# Autodesk Inventor assembly: Ensamblaje
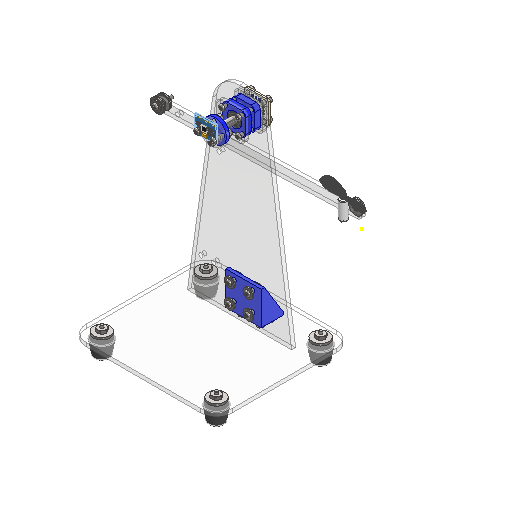
[picture p0: Inventor's stored thumbnail of the model, 512x512]
Saved by Autodesk Inventor 2025.3 (Build 293356000, 356)
## iProperties
Created: 2025-11-11
Part Number: Ensamblaje
Document SubType Name: Assembly
Designer: Gabriel Bojaca
Author: Gabriel Bojaca
## Documents named in this file (28)
- C:\Users\Gabriel Bojaca\Documents\Inventor\TDC\Ensamblaje.iam
- C:\Users\Gabriel Bojaca\Documents\Inventor\TDC\Acople_eje.ipt
- C:\Users\Gabriel Bojaca\Documents\Inventor\TDC\Base.ipt
- C:\Users\Gabriel Bojaca\Documents\Inventor\TDC\Chumacera.ipt
- C:\Users\Gabriel Bojaca\Documents\Inventor\TDC\Columna.ipt
- C:\Users\Gabriel Bojaca\Documents\Inventor\TDC\Escuadra.ipt
- C:\Users\Gabriel Bojaca\Documents\Inventor\TDC\Tope_rodamiento.ipt
- C:\Users\Gabriel Bojaca\Documents\Inventor\TDC\MR126ZZ-6x12x4mm.ipt
- C:\Users\Gabriel Bojaca\Documents\Inventor\TDC\Pendulo.ipt
- C:\Users\Gabriel Bojaca\Documents\Inventor\TDC\eje.ipt
- C:\Users\Gabriel Bojaca\Documents\Inventor\TDC\AS5600_magnetic_encoder\AS5600_magnetic_encoder\AS5600_magnetic_encoder.ipt
- C:\Users\Gabriel Bojaca\Documents\Inventor\TDC\Separador.ipt
- C:\Users\Gabriel Bojaca\Documents\Inventor\TDC\iman.ipt
- C:\Users\Gabriel Bojaca\Documents\Inventor\TDC\MPU_6050\MPU_6050\MPU_6050.ipt
- C:\Users\Gabriel Bojaca\Documents\Inventor\TDC\Coreless_Motor_716\Coreless_Motor_716\Coreless_Motor_716.ipt
- C:\Users\Gabriel Bojaca\Documents\Inventor\Content Center Files\R2025\en-US\ANSI B18.3.4M(1)\ANSI B18.3.4M - M3 x 0.5 x 30(2).ipt
- C:\Users\Gabriel Bojaca\Documents\Inventor\Content Center Files\R2025\en-US\ANSI B18.2.4.2M\ANSI B18.2.4.2M - M3x0,5 - 5,5.ipt
- C:\Users\Gabriel Bojaca\Documents\Inventor\Content Center Files\R2025\en-US\ANSI B18.3.4M(1)\ANSI B18.3.4M - M3 x 0.5 x 10(2).ipt
- C:\Users\Gabriel Bojaca\Documents\Inventor\Content Center Files\R2025\en-US\ANSI B18.3.4M(1)\ANSI B18.3.4M - M3 x 0.5 x 16(2).ipt
- C:\Users\Gabriel Bojaca\Documents\Inventor\TDC\Arandela_3_16.ipt
- C:\Users\Gabriel Bojaca\Documents\Inventor\TDC\Arandela_1_8.ipt
- C:\Users\Gabriel Bojaca\Documents\Inventor\TDC\Tuerca_M3.ipt
- C:\Users\Gabriel Bojaca\Documents\Inventor\Content Center Files\R2025\en-US\ANSI B18.3.4M(1)\ANSI B18.3.4M - M3 x 0.5 x 12(2).ipt
- C:\Users\Gabriel Bojaca\Documents\Inventor\TDC\Patas_para_licuadora.ipt
- C:\Users\Gabriel Bojaca\Documents\Inventor\Content Center Files\R2025\en-US\ANSI B18.6.3(48)\ANSI B18.6.3 - 4-40 x 3_4(7).ipt
- C:\Users\Gabriel Bojaca\Documents\Inventor\Content Center Files\R2025\en-US\ANSI B18.2.2(06)\ANSI B18.2.2 - 5 - 44(06).ipt
- C:\Users\Gabriel Bojaca\Documents\Inventor\Content Center Files\R2025\en-US\ASTM F436(1)\ASTM F436 - 1_4(1).ipt
- C:\Users\Gabriel Bojaca\Documents\Inventor\TDC\PROPELLER - 8x4.5 CW\cw_2blades.ipt
## Components (90 placed, 27 different names)
1. Acople_eje:1 — Mate:26, Mate:27, Mate:28, Mate:29, Mate:74, Mate:76, Mate:77, Mate:81, Mate:86
2. Base:1 — Mate:1, Mate:8, Mate:9, Mate:10, Mate:144, Mate:153, Mate:154, Mate:155, Mate:156, Mate:157, Mate:158, Mate:159, Mate:162, Mate:175, Mate:176, Mate:177, Mate:179, Mate:180, Mate:183
3. Chumacera:1 — Mate:12, Flush:1, Mate:16, Mate:20, Mate:22
4. Columna:1 — Mate:5, Mate:6, Mate:7, Mate:13, Mate:14, Mate:15, Mate:16, Mate:54, Mate:115, Mate:133, Mate:134, Mate:135, Mate:136
5. Escuadra:1 — Mate:5, Mate:6, Mate:7, Mate:8, Mate:9, Mate:10, Mate:116, Mate:117, Mate:137, Mate:142, Mate:143, Mate:148, Mate:149, Mate:150, Mate:151, Mate:152
6. Tope_rodamiento:1 — Mate:20, Mate:21, Mate:22, Mate:23, Mate:54, Mate:55, Mate:56, Mate:62, Mate:63, Mate:65, Mate:66, Mate:69, Mate:70
7. Chumacera:2 — Mate:11, Flush:2, Mate:15, Mate:18, Mate:19
8. MR126ZZ-6x12x4mm:1 — Mate:12, Flush:1, Mate:13, Mate:21, Mate:31
9. MR126ZZ-6x12x4mm:2 — Mate:11, Flush:2, Mate:14, Mate:17
10. Tope_rodamiento:2 — Mate:17, Mate:18, Mate:19, Mate:23, Mate:32, Mate:33, Mate:34, Mate:35, Mate:36, Mate:37, Mate:38, Mate:39, Mate:40, Mate:41
11. Pendulo:1 — Mate:26, Mate:27, Mate:28, Mate:30, Mate:46, Mate:47, Mate:48, Mate:49, Mate:186, Mate:53, Mate:72, Mate:73, Mate:78, Mate:87, Mate:94, Mate:95, Mate:96, Mate:108, Mate:109
12. eje:1 — Mate:29, Mate:30, Mate:31, Mate:43, Mate:44
13. AS5600_magnetic_encoder:1 — Mate:32, Mate:33, Mate:42, Mate:45, Mate:58, Mate:64, Mate:67, Mate:68
14. Separador:1 — Mate:35, Mate:40
15. Separador:2 — Mate:36, Mate:41, Mate:42
16. Separador:3 — Mate:34, Mate:38
17. Separador:4 — Mate:37, Mate:39
18. iman:1 — Mate:43, Mate:44, Mate:45
19. MPU_6050:1 — Mate:50, Mate:51, Mate:52, Mate:80, Mate:82, Mate:84, Mate:85
20. Separador:5 — Mate:46, Mate:48, Mate:50, Mate:52
21. Separador:6 — Mate:47, Mate:49, Mate:51
22. Coreless_Motor_716:1 — Mate:186, Mate:53, Mate:87, Mate:184, Mate:185
23. Broached Hexagon Socket Button Head Cap Screw - Metric M3 x 0.5 x 30:2 — Mate:55, Mate:56, Mate:57
24. ANSI B18.2.4.2M M3x0,5:1 — Mate:57, Mate:58
25. Broached Hexagon Socket Button Head Cap Screw - Metric M3 x 0.5 x 30:3 — Mate:69, Mate:70
26. ANSI B18.2.4.2M M3x0,5:2 — Mate:68
27. Broached Hexagon Socket Button Head Cap Screw - Metric M3 x 0.5 x 30:4 — Mate:62, Mate:63
28. ANSI B18.2.4.2M M3x0,5:3 — Mate:64
29. Broached Hexagon Socket Button Head Cap Screw - Metric M3 x 0.5 x 30:5 — Mate:65, Mate:66
30. ANSI B18.2.4.2M M3x0,5:4 — Mate:67
31. Broached Hexagon Socket Button Head Cap Screw - Metric M3 x 0.5 x 10:1 — Mate:72, Mate:73
32. ANSI B18.2.4.2M M3x0,5:5 — Mate:74
33. Broached Hexagon Socket Button Head Cap Screw - Metric M3 x 0.5 x 10:2 — Mate:76, Mate:78
34. ANSI B18.2.4.2M M3x0,5:6 — Mate:77
35. Broached Hexagon Socket Button Head Cap Screw - Metric M3 x 0.5 x 16:1 — Mate:80, Mate:82
36. ANSI B18.2.4.2M M3x0,5:7 — Mate:81
37. Broached Hexagon Socket Button Head Cap Screw - Metric M3 x 0.5 x 16:2 — Mate:84, Mate:85
38. ANSI B18.2.4.2M M3x0,5:8 — Mate:86
39. Broached Hexagon Socket Button Head Cap Screw - Metric M3 x 0.5 x 16:3 — Mate:88, Mate:89, Mate:91, Mate:93, Mate:94, Mate:97, Mate:98, Mate:101, Mate:102
40. Arandela_3_16:1 — Mate:96, Mate:97, Mate:99
41. Arandela_1_8:1 — Mate:100, Mate:101, Mate:103
42. Arandela_3_16:2 — Mate:89, Mate:90, Mate:92
43. Arandela_1_8:2 — Mate:88, Mate:90, Mate:91
44. Tuerca_M3:2 — Mate:102, Mate:103
45. Arandela_3_16:3 — Mate:98, Mate:99, Mate:100
46. Arandela_3_16:4 — Mate:92, Mate:93, Mate:95
47. Arandela_3_16:5 — Mate:104, Mate:106, Mate:108, Mate:109
48. Arandela_3_16:6 — Mate:104, Mate:105, Mate:107
49. Arandela_3_16:7 — Mate:105, Mate:106, Mate:107
50. Broached Hexagon Socket Button Head Cap Screw - Metric M3 x 0.5 x 12:1 — Mate:117
51. Arandela_1_8:3 — Mate:116
52. Arandela_1_8:4 — Mate:115
53. Tuerca_M3:3
54. Broached Hexagon Socket Button Head Cap Screw - Metric M3 x 0.5 x 12:2 — Mate:134
55. Arandela_1_8:5 — Flush:6, Mate:137
56. Arandela_1_8:6 — Flush:4, Mate:133
57. Tuerca_M3:4
58. Broached Hexagon Socket Button Head Cap Screw - Metric M3 x 0.5 x 12:3 — Mate:135
59. Arandela_1_8:7 — Flush:6, Flush:7
60. Arandela_1_8:8 — Flush:4, Flush:5
61. Tuerca_M3:5
62. Broached Hexagon Socket Button Head Cap Screw - Metric M3 x 0.5 x 12:4 — Mate:136
63. Arandela_1_8:9 — Flush:7
64. Arandela_1_8:10 — Flush:5
65. Tuerca_M3:6
66. Broached Hexagon Socket Button Head Cap Screw - Metric M3 x 0.5 x 10:3 — Mate:142, Mate:143
67. Tuerca_M3:7 — Mate:144
68. Broached Hexagon Socket Button Head Cap Screw - Metric M3 x 0.5 x 10:4 — Mate:148, Mate:149
69. Tuerca_M3:8 — Flush:9, Flush:10
70. Broached Hexagon Socket Button Head Cap Screw - Metric M3 x 0.5 x 10:5 — Flush:8, Mate:150, Mate:152
71. Tuerca_M3:9 — Flush:9
72. Broached Hexagon Socket Button Head Cap Screw - Metric M3 x 0.5 x 10:6 — Flush:8, Mate:151
73. Tuerca_M3:10 — Flush:10, Mate:153
74. Patas_para_licuadora:1 — Mate:154, Mate:155
75. Patas_para_licuadora:2 — Mate:156, Flush:11, Mate:160, Mate:161
76. Patas_para_licuadora:3 — Mate:157, Flush:12, Mate:159, Mate:182
77. Patas_para_licuadora:4 — Mate:158, Flush:11, Flush:12, Mate:181
78. Slotted Hex Head Machine Screw - Inch 4-40 x 3/4:1 — Mate:160, Mate:161, Mate:163, Mate:165
79. Hex Machine Screw Nut - Inch 5 - 44:1 — Mate:164, Mate:165
80. Circular Washer (Inch) 1/4:1 — Mate:162, Mate:163, Mate:164
81. Slotted Hex Head Machine Screw - Inch 4-40 x 3/4:2 — Mate:175, Mate:182
82. Hex Machine Screw Nut - Inch 5 - 44:2
83. Circular Washer (Inch) 1/4:2 — Mate:183
84. Slotted Hex Head Machine Screw - Inch 4-40 x 3/4:3 — Flush:14, Mate:177, Mate:181
85. Hex Machine Screw Nut - Inch 5 - 44:3
86. Circular Washer (Inch) 1/4:3 — Mate:179
87. Slotted Hex Head Machine Screw - Inch 4-40 x 3/4:4 — Flush:14, Mate:176
88. Hex Machine Screw Nut - Inch 5 - 44:4
89. Circular Washer (Inch) 1/4:4 — Mate:180
90. cw_2blades:1 — Mate:184, Mate:185
## Relationships (189: Mate 177, Flush 12)
- Mate:1: Base:1
- Mate:5: Columna:1 ↔ Escuadra:1
- Mate:6: Columna:1 ↔ Escuadra:1
- Mate:7: Columna:1 ↔ Escuadra:1
- Mate:8: Base:1 ↔ Escuadra:1
- Mate:9: Base:1 ↔ Escuadra:1
- Mate:10: Base:1 ↔ Escuadra:1
- Mate:11: Chumacera:2 ↔ MR126ZZ-6x12x4mm:2
- Mate:12: Chumacera:1 ↔ MR126ZZ-6x12x4mm:1
- Flush:1 (0.5 mm): Chumacera:1 ↔ MR126ZZ-6x12x4mm:1
- Flush:2 (-0.5 mm): Chumacera:2 ↔ MR126ZZ-6x12x4mm:2
- Mate:13: Columna:1 ↔ MR126ZZ-6x12x4mm:1
- Mate:14: Columna:1 ↔ MR126ZZ-6x12x4mm:2
- Mate:15: Columna:1 ↔ Chumacera:2
- Mate:16: Chumacera:1 ↔ Columna:1
- Mate:17: MR126ZZ-6x12x4mm:2 ↔ Tope_rodamiento:2
- Mate:18: Chumacera:2 ↔ Tope_rodamiento:2
- Mate:19: Chumacera:2 ↔ Tope_rodamiento:2
- Mate:20: Chumacera:1 ↔ Tope_rodamiento:1
- Mate:21: Tope_rodamiento:1 ↔ MR126ZZ-6x12x4mm:1
- Mate:22: Chumacera:1 ↔ Tope_rodamiento:1
- Mate:23: Tope_rodamiento:1 ↔ Tope_rodamiento:2
- Mate:26: Acople_eje:1 ↔ Pendulo:1
- Mate:27: Acople_eje:1 ↔ Pendulo:1
- Mate:28: Acople_eje:1 ↔ Pendulo:1
- Mate:29: Acople_eje:1 ↔ eje:1
- Mate:30: Pendulo:1 ↔ eje:1
- Mate:31: MR126ZZ-6x12x4mm:1 ↔ eje:1
- Mate:32: Tope_rodamiento:2 ↔ AS5600_magnetic_encoder:1
- Mate:33: Tope_rodamiento:2 ↔ AS5600_magnetic_encoder:1
- Mate:34: Tope_rodamiento:2 ↔ Separador:3
- Mate:35: Tope_rodamiento:2 ↔ Separador:1
- Mate:36: Tope_rodamiento:2 ↔ Separador:2
- Mate:37: Tope_rodamiento:2 ↔ Separador:4
- Mate:38: Tope_rodamiento:2 ↔ Separador:3
- Mate:39: Tope_rodamiento:2 ↔ Separador:4
- Mate:40: Tope_rodamiento:2 ↔ Separador:1
- Mate:41: Tope_rodamiento:2 ↔ Separador:2
- Mate:42: AS5600_magnetic_encoder:1 ↔ Separador:2
- Mate:43: eje:1 ↔ iman:1
- Mate:44: eje:1 ↔ iman:1
- Mate:45 (0.5 mm): AS5600_magnetic_encoder:1 ↔ iman:1
- Mate:46: Pendulo:1 ↔ Separador:5
- Mate:47: Pendulo:1 ↔ Separador:6
- Mate:48: Pendulo:1 ↔ Separador:5
- Mate:49: Pendulo:1 ↔ Separador:6
- Mate:50: MPU_6050:1 ↔ Separador:5
- Mate:51: MPU_6050:1 ↔ Separador:6
- Mate:52: MPU_6050:1 ↔ Separador:5
- Mate:186 (-13 mm): Pendulo:1 ↔ Coreless_Motor_716:1
- Mate:53 (3.5 mm): Pendulo:1 ↔ Coreless_Motor_716:1
- Mate:54: Columna:1 ↔ Tope_rodamiento:1
- Mate:55: Tope_rodamiento:1 ↔ Broached Hexagon Socket Button Head Cap Screw - Metric M3 x 0.5 x 30:2
- Mate:56: Tope_rodamiento:1 ↔ Broached Hexagon Socket Button Head Cap Screw - Metric M3 x 0.5 x 30:2
- Mate:57: Broached Hexagon Socket Button Head Cap Screw - Metric M3 x 0.5 x 30:2 ↔ ANSI B18.2.4.2M M3x0,5:1
- Mate:58: AS5600_magnetic_encoder:1 ↔ ANSI B18.2.4.2M M3x0,5:1
- [Mate]: Broached Hexagon Socket Button Head Cap Screw - Metric M3 x 0.5 x 30:3 ↔ ANSI B18.2.4.2M M3x0,5:2
- [Mate]: Broached Hexagon Socket Button Head Cap Screw - Metric M3 x 0.5 x 30:4 ↔ ANSI B18.2.4.2M M3x0,5:3
- [Mate]: Broached Hexagon Socket Button Head Cap Screw - Metric M3 x 0.5 x 30:5 ↔ ANSI B18.2.4.2M M3x0,5:4
- Mate:62: Tope_rodamiento:1 ↔ Broached Hexagon Socket Button Head Cap Screw - Metric M3 x 0.5 x 30:4
- Mate:63: Tope_rodamiento:1 ↔ Broached Hexagon Socket Button Head Cap Screw - Metric M3 x 0.5 x 30:4
- Mate:64: AS5600_magnetic_encoder:1 ↔ ANSI B18.2.4.2M M3x0,5:3
- Mate:65: Tope_rodamiento:1 ↔ Broached Hexagon Socket Button Head Cap Screw - Metric M3 x 0.5 x 30:5
- Mate:66: Tope_rodamiento:1 ↔ Broached Hexagon Socket Button Head Cap Screw - Metric M3 x 0.5 x 30:5
- Mate:67: AS5600_magnetic_encoder:1 ↔ ANSI B18.2.4.2M M3x0,5:4
- Mate:68: AS5600_magnetic_encoder:1 ↔ ANSI B18.2.4.2M M3x0,5:2
- Mate:69: Tope_rodamiento:1 ↔ Broached Hexagon Socket Button Head Cap Screw - Metric M3 x 0.5 x 30:3
- Mate:70: Tope_rodamiento:1 ↔ Broached Hexagon Socket Button Head Cap Screw - Metric M3 x 0.5 x 30:3
- [Mate]: Broached Hexagon Socket Button Head Cap Screw - Metric M3 x 0.5 x 10:1 ↔ ANSI B18.2.4.2M M3x0,5:5
- Mate:72: Pendulo:1 ↔ Broached Hexagon Socket Button Head Cap Screw - Metric M3 x 0.5 x 10:1
- Mate:73: Pendulo:1 ↔ Broached Hexagon Socket Button Head Cap Screw - Metric M3 x 0.5 x 10:1
- Mate:74: Acople_eje:1 ↔ ANSI B18.2.4.2M M3x0,5:5
- [Mate]: Broached Hexagon Socket Button Head Cap Screw - Metric M3 x 0.5 x 10:2 ↔ ANSI B18.2.4.2M M3x0,5:6
- Mate:76: Acople_eje:1 ↔ Broached Hexagon Socket Button Head Cap Screw - Metric M3 x 0.5 x 10:2
- Mate:77: Acople_eje:1 ↔ ANSI B18.2.4.2M M3x0,5:6
- Mate:78: Pendulo:1 ↔ Broached Hexagon Socket Button Head Cap Screw - Metric M3 x 0.5 x 10:2
- [Mate]: Broached Hexagon Socket Button Head Cap Screw - Metric M3 x 0.5 x 16:1 ↔ ANSI B18.2.4.2M M3x0,5:7
- Mate:80: MPU_6050:1 ↔ Broached Hexagon Socket Button Head Cap Screw - Metric M3 x 0.5 x 16:1
- Mate:81: Acople_eje:1 ↔ ANSI B18.2.4.2M M3x0,5:7
- Mate:82: MPU_6050:1 ↔ Broached Hexagon Socket Button Head Cap Screw - Metric M3 x 0.5 x 16:1
- [Mate]: Broached Hexagon Socket Button Head Cap Screw - Metric M3 x 0.5 x 16:2 ↔ ANSI B18.2.4.2M M3x0,5:8
- Mate:84: MPU_6050:1 ↔ Broached Hexagon Socket Button Head Cap Screw - Metric M3 x 0.5 x 16:2
- Mate:85: MPU_6050:1 ↔ Broached Hexagon Socket Button Head Cap Screw - Metric M3 x 0.5 x 16:2
- Mate:86: Acople_eje:1 ↔ ANSI B18.2.4.2M M3x0,5:8
- Mate:87 (14.5 mm): Pendulo:1 ↔ Coreless_Motor_716:1
- Mate:88: Broached Hexagon Socket Button Head Cap Screw - Metric M3 x 0.5 x 16:3 ↔ Arandela_1_8:2
- Mate:89: Broached Hexagon Socket Button Head Cap Screw - Metric M3 x 0.5 x 16:3 ↔ Arandela_3_16:2
- Mate:90: Arandela_3_16:2 ↔ Arandela_1_8:2
- Mate:91: Broached Hexagon Socket Button Head Cap Screw - Metric M3 x 0.5 x 16:3 ↔ Arandela_1_8:2
- Mate:92: Arandela_3_16:2 ↔ Arandela_3_16:4
- Mate:93: Broached Hexagon Socket Button Head Cap Screw - Metric M3 x 0.5 x 16:3 ↔ Arandela_3_16:4
- Mate:94: Pendulo:1 ↔ Broached Hexagon Socket Button Head Cap Screw - Metric M3 x 0.5 x 16:3
- Mate:95: Pendulo:1 ↔ Arandela_3_16:4
- Mate:96: Pendulo:1 ↔ Arandela_3_16:1
- Mate:97: Broached Hexagon Socket Button Head Cap Screw - Metric M3 x 0.5 x 16:3 ↔ Arandela_3_16:1
- Mate:98: Broached Hexagon Socket Button Head Cap Screw - Metric M3 x 0.5 x 16:3 ↔ Arandela_3_16:3
- Mate:99: Arandela_3_16:1 ↔ Arandela_3_16:3
- Mate:100: Arandela_1_8:1 ↔ Arandela_3_16:3
- Mate:101: Broached Hexagon Socket Button Head Cap Screw - Metric M3 x 0.5 x 16:3 ↔ Arandela_1_8:1
- Mate:102: Broached Hexagon Socket Button Head Cap Screw - Metric M3 x 0.5 x 16:3 ↔ Tuerca_M3:2
- Mate:103: Arandela_1_8:1 ↔ Tuerca_M3:2
- Mate:104: Arandela_3_16:5 ↔ Arandela_3_16:6
- Mate:105: Arandela_3_16:6 ↔ Arandela_3_16:7
- Mate:106: Arandela_3_16:5 ↔ Arandela_3_16:7
- Mate:107: Arandela_3_16:6 ↔ Arandela_3_16:7
- Mate:108: Pendulo:1 ↔ Arandela_3_16:5
- Mate:109: Pendulo:1 ↔ Arandela_3_16:5
- [Mate]: Broached Hexagon Socket Button Head Cap Screw - Metric M3 x 0.5 x 12:1 ↔ Arandela_1_8:4
- [Mate]: Broached Hexagon Socket Button Head Cap Screw - Metric M3 x 0.5 x 12:1 ↔ Arandela_1_8:4
- [Mate]: Broached Hexagon Socket Button Head Cap Screw - Metric M3 x 0.5 x 12:1 ↔ Arandela_1_8:3
- [Mate]: Broached Hexagon Socket Button Head Cap Screw - Metric M3 x 0.5 x 12:1 ↔ Tuerca_M3:3
- [Mate]: Arandela_1_8:3 ↔ Tuerca_M3:3
- Mate:115: Columna:1 ↔ Arandela_1_8:4
- Mate:116: Escuadra:1 ↔ Arandela_1_8:3
- Mate:117: Escuadra:1 ↔ Broached Hexagon Socket Button Head Cap Screw - Metric M3 x 0.5 x 12:1
- [Mate]: Broached Hexagon Socket Button Head Cap Screw - Metric M3 x 0.5 x 12:2 ↔ Arandela_1_8:6
- [Mate]: Broached Hexagon Socket Button Head Cap Screw - Metric M3 x 0.5 x 12:2 ↔ Arandela_1_8:6
- [Mate]: Broached Hexagon Socket Button Head Cap Screw - Metric M3 x 0.5 x 12:2 ↔ Arandela_1_8:5
- [Mate]: Broached Hexagon Socket Button Head Cap Screw - Metric M3 x 0.5 x 12:2 ↔ Tuerca_M3:4
- [Mate]: Arandela_1_8:5 ↔ Tuerca_M3:4
- [Mate]: Broached Hexagon Socket Button Head Cap Screw - Metric M3 x 0.5 x 12:3 ↔ Arandela_1_8:8
- [Mate]: Broached Hexagon Socket Button Head Cap Screw - Metric M3 x 0.5 x 12:3 ↔ Arandela_1_8:8
- [Mate]: Broached Hexagon Socket Button Head Cap Screw - Metric M3 x 0.5 x 12:3 ↔ Arandela_1_8:7
- [Mate]: Broached Hexagon Socket Button Head Cap Screw - Metric M3 x 0.5 x 12:3 ↔ Tuerca_M3:5
- [Mate]: Arandela_1_8:7 ↔ Tuerca_M3:5
- [Mate]: Broached Hexagon Socket Button Head Cap Screw - Metric M3 x 0.5 x 12:4 ↔ Arandela_1_8:10
- [Mate]: Broached Hexagon Socket Button Head Cap Screw - Metric M3 x 0.5 x 12:4 ↔ Arandela_1_8:10
- [Mate]: Broached Hexagon Socket Button Head Cap Screw - Metric M3 x 0.5 x 12:4 ↔ Arandela_1_8:9
- [Mate]: Broached Hexagon Socket Button Head Cap Screw - Metric M3 x 0.5 x 12:4 ↔ Tuerca_M3:6
- [Mate]: Arandela_1_8:9 ↔ Tuerca_M3:6
- Flush:4: Arandela_1_8:6 ↔ Arandela_1_8:8
- Flush:5: Arandela_1_8:8 ↔ Arandela_1_8:10
- Flush:6: Arandela_1_8:5 ↔ Arandela_1_8:7
- Flush:7: Arandela_1_8:7 ↔ Arandela_1_8:9
- Mate:133: Columna:1 ↔ Arandela_1_8:6
- Mate:134: Columna:1 ↔ Broached Hexagon Socket Button Head Cap Screw - Metric M3 x 0.5 x 12:2
- Mate:135: Columna:1 ↔ Broached Hexagon Socket Button Head Cap Screw - Metric M3 x 0.5 x 12:3
- Mate:136: Columna:1 ↔ Broached Hexagon Socket Button Head Cap Screw - Metric M3 x 0.5 x 12:4
- Mate:137: Escuadra:1 ↔ Arandela_1_8:5
- [Mate]: Broached Hexagon Socket Button Head Cap Screw - Metric M3 x 0.5 x 10:3 ↔ Tuerca_M3:7
- Mate:142: Escuadra:1 ↔ Broached Hexagon Socket Button Head Cap Screw - Metric M3 x 0.5 x 10:3
- Mate:143: Escuadra:1 ↔ Broached Hexagon Socket Button Head Cap Screw - Metric M3 x 0.5 x 10:3
- Mate:144: Base:1 ↔ Tuerca_M3:7
- [Mate]: Broached Hexagon Socket Button Head Cap Screw - Metric M3 x 0.5 x 10:4 ↔ Tuerca_M3:8
- [Mate]: Broached Hexagon Socket Button Head Cap Screw - Metric M3 x 0.5 x 10:5 ↔ Tuerca_M3:9
- [Mate]: Broached Hexagon Socket Button Head Cap Screw - Metric M3 x 0.5 x 10:6 ↔ Tuerca_M3:10
- Mate:148: Escuadra:1 ↔ Broached Hexagon Socket Button Head Cap Screw - Metric M3 x 0.5 x 10:4
- Flush:8: Broached Hexagon Socket Button Head Cap Screw - Metric M3 x 0.5 x 10:5 ↔ Broached Hexagon Socket Button Head Cap Screw - Metric M3 x 0.5 x 10:6
- Mate:149: Escuadra:1 ↔ Broached Hexagon Socket Button Head Cap Screw - Metric M3 x 0.5 x 10:4
- Mate:150: Escuadra:1 ↔ Broached Hexagon Socket Button Head Cap Screw - Metric M3 x 0.5 x 10:5
- Mate:151: Escuadra:1 ↔ Broached Hexagon Socket Button Head Cap Screw - Metric M3 x 0.5 x 10:6
- Mate:152: Escuadra:1 ↔ Broached Hexagon Socket Button Head Cap Screw - Metric M3 x 0.5 x 10:5
- Flush:9: Tuerca_M3:8 ↔ Tuerca_M3:9
- Flush:10: Tuerca_M3:8 ↔ Tuerca_M3:10
- Mate:153: Base:1 ↔ Tuerca_M3:10
- Mate:154: Base:1 ↔ Patas_para_licuadora:1
- Mate:155: Base:1 ↔ Patas_para_licuadora:1
- Mate:156: Base:1 ↔ Patas_para_licuadora:2
- Mate:157: Base:1 ↔ Patas_para_licuadora:3
- Mate:158: Base:1 ↔ Patas_para_licuadora:4
- Flush:11: Patas_para_licuadora:2 ↔ Patas_para_licuadora:4
- Flush:12: Patas_para_licuadora:3 ↔ Patas_para_licuadora:4
- Mate:159: Base:1 ↔ Patas_para_licuadora:3
- Mate:160: Patas_para_licuadora:2 ↔ Slotted Hex Head Machine Screw - Inch 4-40 x 3/4:1
- Mate:161: Patas_para_licuadora:2 ↔ Slotted Hex Head Machine Screw - Inch 4-40 x 3/4:1
- Mate:162: Base:1 ↔ Circular Washer (Inch) 1/4:1
- Mate:163: Slotted Hex Head Machine Screw - Inch 4-40 x 3/4:1 ↔ Circular Washer (Inch) 1/4:1
- Mate:164: Hex Machine Screw Nut - Inch 5 - 44:1 ↔ Circular Washer (Inch) 1/4:1
- Mate:165: Slotted Hex Head Machine Screw - Inch 4-40 x 3/4:1 ↔ Hex Machine Screw Nut - Inch 5 - 44:1
- [Mate]: Slotted Hex Head Machine Screw - Inch 4-40 x 3/4:2 ↔ Circular Washer (Inch) 1/4:2
- [Mate]: Hex Machine Screw Nut - Inch 5 - 44:2 ↔ Circular Washer (Inch) 1/4:2
- [Mate]: Slotted Hex Head Machine Screw - Inch 4-40 x 3/4:2 ↔ Hex Machine Screw Nut - Inch 5 - 44:2
- [Mate]: Slotted Hex Head Machine Screw - Inch 4-40 x 3/4:3 ↔ Circular Washer (Inch) 1/4:3
- [Mate]: Hex Machine Screw Nut - Inch 5 - 44:3 ↔ Circular Washer (Inch) 1/4:3
- [Mate]: Slotted Hex Head Machine Screw - Inch 4-40 x 3/4:3 ↔ Hex Machine Screw Nut - Inch 5 - 44:3
- [Mate]: Slotted Hex Head Machine Screw - Inch 4-40 x 3/4:4 ↔ Circular Washer (Inch) 1/4:4
- [Mate]: Hex Machine Screw Nut - Inch 5 - 44:4 ↔ Circular Washer (Inch) 1/4:4
- [Mate]: Slotted Hex Head Machine Screw - Inch 4-40 x 3/4:4 ↔ Hex Machine Screw Nut - Inch 5 - 44:4
- Flush:14: Slotted Hex Head Machine Screw - Inch 4-40 x 3/4:3 ↔ Slotted Hex Head Machine Screw - Inch 4-40 x 3/4:4
- Mate:175: Base:1 ↔ Slotted Hex Head Machine Screw - Inch 4-40 x 3/4:2
- Mate:176: Base:1 ↔ Slotted Hex Head Machine Screw - Inch 4-40 x 3/4:4
- Mate:177: Base:1 ↔ Slotted Hex Head Machine Screw - Inch 4-40 x 3/4:3
- Mate:179: Base:1 ↔ Circular Washer (Inch) 1/4:3
- Mate:180: Base:1 ↔ Circular Washer (Inch) 1/4:4
- Mate:181: Patas_para_licuadora:4 ↔ Slotted Hex Head Machine Screw - Inch 4-40 x 3/4:3
- Mate:182: Patas_para_licuadora:3 ↔ Slotted Hex Head Machine Screw - Inch 4-40 x 3/4:2
- Mate:183: Base:1 ↔ Circular Washer (Inch) 1/4:2
- Mate:184: Coreless_Motor_716:1 ↔ cw_2blades:1
- Mate:185 (-4 mm): Coreless_Motor_716:1 ↔ cw_2blades:1
## Named parameters: d63_d61 = 0 mm, d64_d63_d61 = 0 mm, d65_d63_d61 = 0 mm, d75_d61 = 0 mm, d79_d75_d61 = 0 mm, d83_d75_d61 = 0 mm, d87_d83_d75_d61 = 0 mm, d114_d92 = 0 mm, d115_d95 = 0 mm, d116_d105 = 0 mm, d117_d106 = 0 mm, d118_d107 = 0 mm, d122_d92 = 0 mm, d123_d95 = 0 mm, d124_d105 = 0 mm, d125_d106 = 0 mm, d126_d107 = 0 mm, d127_d92 = 0 mm, d128_d95 = 0 mm, d129_d105 = 0 mm, d130_d106 = 0 mm, d131_d107 = 0 mm, d132_d92 = 0 mm, d133_d95 = 0 mm, d134_d105 = 0 mm, d135_d106 = 0 mm, d136_d107 = 0 mm, d149_d125_d106 = 0 mm, d154_d149_d125_d106 = 0 mm, d155_d149_d125_d106 = 0 mm, d156_d149_d125_d106 = 0 mm, d180_d177 = 0 mm, d181_d178 = 0 mm, d182_d179 = 0 mm, d183_d177 = 0 mm, d184_d178 = 0 mm, d185_d179 = 0 mm, d186_d177 = 0 mm, d187_d178 = 0 mm, d188_d179 = 0 mm
